# Autodesk Inventor assembly: Cockpit
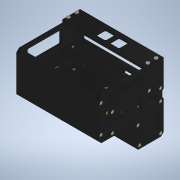
[picture p0: Inventor's stored thumbnail of the model, 180x180]
Saved by Autodesk Inventor 2020 (Build 240168000, 168)
## iProperties
Created: 2022-01-06
Part Number: Cockpit
Document SubType Name: Assembly
Designer: Masato Kubotera
Mass: 580.21 g
Surface Area: 2312.67 cm^2
Volume: 391.499 cm^3
Density: 1.48202 g/cm^3
Author: Masato Kubotera
## Documents named in this file (17)
- C:\Users\MasatoKubotera\Documents\Inventor\OpenPlatform_ver3_0 - prototype\UpperBody\Cockpit\Cockpit.iam
- C:\Users\MasatoKubotera\Documents\Inventor\OpenPlatform_ver3_0 - prototype\ReadyMade\Battery\HP-G830C2800S3.ipt
- C:\Users\MasatoKubotera\Documents\Inventor\OpenPlatform_ver3_0 - prototype\UpperBody\Cockpit\Cockpit_side_frame.ipt
- C:\Users\MasatoKubotera\Documents\Inventor\OpenPlatform_ver3_0 - prototype\UpperBody\Cockpit\Cockpit_battery_back_boor.ipt
- C:\Users\MasatoKubotera\Documents\Inventor\OpenPlatform_ver3_0 - prototype\UpperBody\Cockpit\Cockpit_battery_bottom_frame.ipt
- C:\Users\MasatoKubotera\Documents\Inventor\OpenPlatform_ver3_0 - prototype\UpperBody\Cockpit\Cockpit_battery_front_frame.ipt
- C:\Users\MasatoKubotera\Documents\Inventor\OpenPlatform_ver3_0 - prototype\UpperBody\Cockpit\Cockpit_circuit_board_frame.ipt
- C:\Users\MasatoKubotera\Documents\Inventor\OpenPlatform_ver3_0 - prototype\UpperBody\Cockpit\Cockpit_front_frame.ipt
- C:\Users\MasatoKubotera\Documents\Inventor\OpenPlatform_ver3_0 - prototype\UpperBody\Cockpit\Cockpit_side_frame_MIR.ipt
- C:\Users\MasatoKubotera\Documents\Inventor\OpenPlatform_ver3_0 - prototype\UpperBody\Cockpit\Cockpit_top_frame.ipt
- C:\Users\MasatoKubotera\Documents\Inventor\OpenPlatform_ver3_0 - prototype\UpperBody\Cockpit\Cockpit_carrier_board_frame.ipt
- C:\Users\MasatoKubotera\Documents\Inventor\OpenPlatform_ver3_0 - prototype\UpperBody\Cockpit\Cockpit_back_frame.ipt
- C:\Users\MasatoKubotera\Documents\Inventor\OpenPlatform_ver3_0 - prototype\ReadyMade\InsertNut\UD-43040.ipt
- C:\Users\MasatoKubotera\Documents\Inventor\OpenPlatform_ver3_0 - prototype\ReadyMade\InsertNut\IRU-304SW.ipt
- C:\Users\MasatoKubotera\Documents\Inventor\OpenPlatform_ver3_0 - prototype\ReadyMade\Neodymium_magnet_Phi3_T3.ipt
- C:\Users\MasatoKubotera\Documents\Inventor\OpenPlatform_ver3_0 - prototype\ReadyMade\Screw\M3-8.ipt
- C:\Users\MasatoKubotera\Documents\Inventor\OpenPlatform_ver3_0 - prototype\ReadyMade\Screw\M3-10.ipt
## Components (79 placed, 16 different names)
1. HP-G830C2800S3:1 — メイト:1, メイト:2, メイト:3
2. Cockpit_side_frame:1 — フラッシュ:1, フラッシュ:2, フラッシュ:3, 挿入:1, 挿入:9, 挿入:10, 挿入:33, 挿入:34, 挿入:35, 挿入:49, 挿入:50, 挿入:53, 挿入:54, 挿入:57, 角度:1, 挿入:59, 挿入:61, 挿入:63, 角度:2, 角度:3, 角度:4, 挿入:65, 挿入:66, メイト:3, 挿入:69, 挿入:70, 挿入:73, 挿入:74, 挿入:77, 挿入:79, 挿入:81, 挿入:83, 挿入:85, 挿入:86
3. Cockpit_battery_back_boor:1 — 挿入:27, 挿入:28, 挿入:39, 挿入:40, 挿入:41, 挿入:42, 挿入:43, 挿入:44, 角度:2
4. Cockpit_battery_bottom_frame:1 — 挿入:25, 挿入:26, メイト:1, 角度:4
5. Cockpit_battery_front_frame:1 — 挿入:23, 挿入:24, 角度:3, メイト:2
6. Cockpit_circuit_board_frame:1 — 挿入:3, 挿入:4, 挿入:5, 挿入:6, 挿入:7, 挿入:8, 挿入:17, 挿入:18, 角度:1
7. Cockpit_front_frame:1 — 挿入:13, 挿入:14, 挿入:15, 挿入:16
8. Cockpit_side_frame_MIR:1 — 挿入:2, 挿入:11, 挿入:12, 挿入:36, 挿入:37, 挿入:38, 挿入:51, 挿入:52, 挿入:55, 挿入:56, 挿入:58, 挿入:60, 挿入:62, 挿入:64, 挿入:67, 挿入:68, 挿入:71, 挿入:72, 挿入:75, 挿入:76, 挿入:78, 挿入:80, 挿入:82, 挿入:84, 挿入:87, 挿入:88
9. Cockpit_top_frame:1 — 挿入:45, 挿入:46, 挿入:47, 挿入:48, 挿入:89, 挿入:90, 挿入:91, 挿入:92
10. Cockpit_carrier_board_frame:1 — 挿入:19, 挿入:20, 挿入:22, 挿入:21
11. M3-8:1 — 挿入:69
12. M3-8:2 — 挿入:70
13. M3-8:3 — 挿入:71
14. M3-8:4 — 挿入:72
15. M3-8:5 — 挿入:73
16. M3-8:6 — 挿入:74
17. M3-8:7 — 挿入:75
18. M3-8:8 — 挿入:76
19. M3-8:9 — 挿入:77
20. M3-8:10 — 挿入:78
21. M3-8:11 — 挿入:79
22. M3-8:12 — 挿入:80
23. M3-8:13 — 挿入:81
24. M3-8:14 — 挿入:82
25. M3-8:15 — 挿入:83
26. M3-8:16 — 挿入:84
27. M3-8:17 — 挿入:85
28. M3-8:18 — 挿入:86
29. M3-8:19 — 挿入:87
30. M3-8:20 — 挿入:88
31. M3-10:1 — 挿入:89
32. M3-10:2 — 挿入:90
33. M3-10:3 — 挿入:91
34. M3-10:4 — 挿入:92
35. Cockpit_back_frame:1 — 挿入:29, 挿入:30, 挿入:31, 挿入:32
36. UD-43040:1 — 挿入:1
37. UD-43040:2 — 挿入:2
38. UD-43040:3 — 挿入:3
39. UD-43040:4 — 挿入:4
40. UD-43040:5 — 挿入:5
41. UD-43040:6 — 挿入:6
42. UD-43040:7 — 挿入:7
43. UD-43040:8 — 挿入:8
44. IRU-304SW:1 — 挿入:9, 挿入:45
45. IRU-304SW:2 — 挿入:10, 挿入:46
46. IRU-304SW:3 — 挿入:11, 挿入:47
47. IRU-304SW:4 — 挿入:12, 挿入:48
48. IRU-304SW:5 — 挿入:13, 挿入:49
49. IRU-304SW:6 — 挿入:14, 挿入:50
50. IRU-304SW:7 — 挿入:15, 挿入:51
51. IRU-304SW:8 — 挿入:16, 挿入:52
52. IRU-304SW:9 — 挿入:17, 挿入:57
53. IRU-304SW:10 — 挿入:18, 挿入:58
54. IRU-304SW:11 — 挿入:19, 挿入:53
55. IRU-304SW:12 — 挿入:20, 挿入:54
56. IRU-304SW:13 — 挿入:21, 挿入:55
57. IRU-304SW:14 — 挿入:22, 挿入:56
58. IRU-304SW:15 — 挿入:23, 挿入:59
59. IRU-304SW:16 — 挿入:24, 挿入:60
60. IRU-304SW:17 — 挿入:25, 挿入:61
61. IRU-304SW:18 — 挿入:26, 挿入:62
62. IRU-304SW:19 — 挿入:27, 挿入:63
63. IRU-304SW:20 — 挿入:28, 挿入:64
64. IRU-304SW:21 — 挿入:29, 挿入:65
65. IRU-304SW:22 — 挿入:30, 挿入:66
66. IRU-304SW:23 — 挿入:31, 挿入:67
67. IRU-304SW:24 — 挿入:32, 挿入:68
68. Neodymium_magnet_Phi3_T3:1 — 挿入:33
69. Neodymium_magnet_Phi3_T3:2 — 挿入:34
70. Neodymium_magnet_Phi3_T3:3 — 挿入:35
71. Neodymium_magnet_Phi3_T3:4 — 挿入:36
72. Neodymium_magnet_Phi3_T3:5 — 挿入:37
73. Neodymium_magnet_Phi3_T3:6 — 挿入:38
74. Neodymium_magnet_Phi3_T3:7 — 挿入:39
75. Neodymium_magnet_Phi3_T3:8 — 挿入:40
76. Neodymium_magnet_Phi3_T3:9 — 挿入:41
77. Neodymium_magnet_Phi3_T3:10 — 挿入:42
78. Neodymium_magnet_Phi3_T3:11 — 挿入:43
79. Neodymium_magnet_Phi3_T3:12 — 挿入:44
## Relationships (102: Insert 92, Angle 4, Flush 3, Mate 3)
- フラッシュ:1 [Flush]: Cockpit_side_frame:1
- フラッシュ:2 [Flush] (67.5 mm): Cockpit_side_frame:1
- フラッシュ:3 [Flush]: Cockpit_side_frame:1
- 挿入:1 [Insert]: Cockpit_side_frame:1 ↔ UD-43040:1
- 挿入:2 [Insert]: Cockpit_side_frame_MIR:1 ↔ UD-43040:2
- 挿入:3 [Insert]: Cockpit_circuit_board_frame:1 ↔ UD-43040:3
- 挿入:4 [Insert]: Cockpit_circuit_board_frame:1 ↔ UD-43040:4
- 挿入:5 [Insert]: Cockpit_circuit_board_frame:1 ↔ UD-43040:5
- 挿入:6 [Insert]: Cockpit_circuit_board_frame:1 ↔ UD-43040:6
- 挿入:7 [Insert]: Cockpit_circuit_board_frame:1 ↔ UD-43040:7
- 挿入:8 [Insert]: Cockpit_circuit_board_frame:1 ↔ UD-43040:8
- 挿入:9 [Insert]: Cockpit_side_frame:1 ↔ IRU-304SW:1
- 挿入:10 [Insert]: Cockpit_side_frame:1 ↔ IRU-304SW:2
- 挿入:11 [Insert]: Cockpit_side_frame_MIR:1 ↔ IRU-304SW:3
- 挿入:12 [Insert]: Cockpit_side_frame_MIR:1 ↔ IRU-304SW:4
- 挿入:13 [Insert]: Cockpit_front_frame:1 ↔ IRU-304SW:5
- 挿入:14 [Insert]: Cockpit_front_frame:1 ↔ IRU-304SW:6
- 挿入:15 [Insert]: Cockpit_front_frame:1 ↔ IRU-304SW:7
- 挿入:16 [Insert]: Cockpit_front_frame:1 ↔ IRU-304SW:8
- 挿入:17 [Insert]: Cockpit_circuit_board_frame:1 ↔ IRU-304SW:9
- 挿入:18 [Insert]: Cockpit_circuit_board_frame:1 ↔ IRU-304SW:10
- 挿入:19 [Insert]: Cockpit_carrier_board_frame:1 ↔ IRU-304SW:11
- 挿入:20 [Insert]: Cockpit_carrier_board_frame:1 ↔ IRU-304SW:12
- 挿入:21 [Insert]: Cockpit_carrier_board_frame:1 ↔ IRU-304SW:13
- 挿入:22 [Insert]: Cockpit_carrier_board_frame:1 ↔ IRU-304SW:14
- 挿入:23 [Insert]: Cockpit_battery_front_frame:1 ↔ IRU-304SW:15
- 挿入:24 [Insert]: Cockpit_battery_front_frame:1 ↔ IRU-304SW:16
- 挿入:25 [Insert]: Cockpit_battery_bottom_frame:1 ↔ IRU-304SW:17
- 挿入:26 [Insert]: Cockpit_battery_bottom_frame:1 ↔ IRU-304SW:18
- 挿入:27 [Insert]: Cockpit_battery_back_boor:1 ↔ IRU-304SW:19
- 挿入:28 [Insert]: Cockpit_battery_back_boor:1 ↔ IRU-304SW:20
- 挿入:29 [Insert]: Cockpit_back_frame:1 ↔ IRU-304SW:21
- 挿入:30 [Insert]: Cockpit_back_frame:1 ↔ IRU-304SW:22
- 挿入:31 [Insert]: Cockpit_back_frame:1 ↔ IRU-304SW:23
- 挿入:32 [Insert]: Cockpit_back_frame:1 ↔ IRU-304SW:24
- 挿入:33 [Insert]: Cockpit_side_frame:1 ↔ Neodymium_magnet_Phi3_T3:1
- 挿入:34 [Insert]: Cockpit_side_frame:1 ↔ Neodymium_magnet_Phi3_T3:2
- 挿入:35 [Insert]: Cockpit_side_frame:1 ↔ Neodymium_magnet_Phi3_T3:3
- 挿入:36 [Insert]: Cockpit_side_frame_MIR:1 ↔ Neodymium_magnet_Phi3_T3:4
- 挿入:37 [Insert]: Cockpit_side_frame_MIR:1 ↔ Neodymium_magnet_Phi3_T3:5
- 挿入:38 [Insert]: Cockpit_side_frame_MIR:1 ↔ Neodymium_magnet_Phi3_T3:6
- 挿入:39 [Insert]: Cockpit_battery_back_boor:1 ↔ Neodymium_magnet_Phi3_T3:7
- 挿入:40 [Insert]: Cockpit_battery_back_boor:1 ↔ Neodymium_magnet_Phi3_T3:8
- 挿入:41 [Insert]: Cockpit_battery_back_boor:1 ↔ Neodymium_magnet_Phi3_T3:9
- 挿入:42 [Insert]: Cockpit_battery_back_boor:1 ↔ Neodymium_magnet_Phi3_T3:10
- 挿入:43 [Insert]: Cockpit_battery_back_boor:1 ↔ Neodymium_magnet_Phi3_T3:11
- 挿入:44 [Insert]: Cockpit_battery_back_boor:1 ↔ Neodymium_magnet_Phi3_T3:12
- 挿入:45 [Insert]: Cockpit_top_frame:1 ↔ IRU-304SW:1
- 挿入:46 [Insert]: Cockpit_top_frame:1 ↔ IRU-304SW:2
- 挿入:47 [Insert]: Cockpit_top_frame:1 ↔ IRU-304SW:3
- 挿入:48 [Insert]: Cockpit_top_frame:1 ↔ IRU-304SW:4
- 挿入:49 [Insert]: Cockpit_side_frame:1 ↔ IRU-304SW:5
- 挿入:50 [Insert]: Cockpit_side_frame:1 ↔ IRU-304SW:6
- 挿入:51 [Insert]: Cockpit_side_frame_MIR:1 ↔ IRU-304SW:7
- 挿入:52 [Insert]: Cockpit_side_frame_MIR:1 ↔ IRU-304SW:8
- 挿入:53 [Insert]: Cockpit_side_frame:1 ↔ IRU-304SW:11
- 挿入:54 [Insert]: Cockpit_side_frame:1 ↔ IRU-304SW:12
- 挿入:55 [Insert]: Cockpit_side_frame_MIR:1 ↔ IRU-304SW:13
- 挿入:56 [Insert]: Cockpit_side_frame_MIR:1 ↔ IRU-304SW:14
- 挿入:57 [Insert]: Cockpit_side_frame:1 ↔ IRU-304SW:9
- 挿入:58 [Insert]: Cockpit_side_frame_MIR:1 ↔ IRU-304SW:10
- 角度:1 [Angle] (0 deg): Cockpit_side_frame:1 ↔ Cockpit_circuit_board_frame:1
- 挿入:59 [Insert]: Cockpit_side_frame:1 ↔ IRU-304SW:15
- 挿入:60 [Insert]: Cockpit_side_frame_MIR:1 ↔ IRU-304SW:16
- 挿入:61 [Insert]: Cockpit_side_frame:1 ↔ IRU-304SW:17
- 挿入:62 [Insert]: Cockpit_side_frame_MIR:1 ↔ IRU-304SW:18
- 挿入:63 [Insert]: Cockpit_side_frame:1 ↔ IRU-304SW:19
- 挿入:64 [Insert]: Cockpit_side_frame_MIR:1 ↔ IRU-304SW:20
- 角度:2 [Angle] (0 deg): Cockpit_side_frame:1 ↔ Cockpit_battery_back_boor:1
- 角度:3 [Angle] (0 deg): Cockpit_side_frame:1 ↔ Cockpit_battery_front_frame:1
- 角度:4 [Angle] (0 deg): Cockpit_side_frame:1 ↔ Cockpit_battery_bottom_frame:1
- 挿入:65 [Insert]: Cockpit_side_frame:1 ↔ IRU-304SW:21
- 挿入:66 [Insert]: Cockpit_side_frame:1 ↔ IRU-304SW:22
- 挿入:67 [Insert]: Cockpit_side_frame_MIR:1 ↔ IRU-304SW:23
- 挿入:68 [Insert]: Cockpit_side_frame_MIR:1 ↔ IRU-304SW:24
- メイト:1 [Mate]: HP-G830C2800S3:1 ↔ Cockpit_battery_bottom_frame:1
- メイト:2 [Mate]: HP-G830C2800S3:1 ↔ Cockpit_battery_front_frame:1
- メイト:3 [Mate]: HP-G830C2800S3:1 ↔ Cockpit_side_frame:1
- 挿入:69 [Insert]: Cockpit_side_frame:1 ↔ M3-8:1
- 挿入:70 [Insert]: Cockpit_side_frame:1 ↔ M3-8:2
- 挿入:71 [Insert]: Cockpit_side_frame_MIR:1 ↔ M3-8:3
- 挿入:72 [Insert]: Cockpit_side_frame_MIR:1 ↔ M3-8:4
- 挿入:73 [Insert]: Cockpit_side_frame:1 ↔ M3-8:5
- 挿入:74 [Insert]: Cockpit_side_frame:1 ↔ M3-8:6
- 挿入:75 [Insert]: Cockpit_side_frame_MIR:1 ↔ M3-8:7
- 挿入:76 [Insert]: Cockpit_side_frame_MIR:1 ↔ M3-8:8
- 挿入:77 [Insert]: Cockpit_side_frame:1 ↔ M3-8:9
- 挿入:78 [Insert]: Cockpit_side_frame_MIR:1 ↔ M3-8:10
- 挿入:79 [Insert]: Cockpit_side_frame:1 ↔ M3-8:11
- 挿入:80 [Insert]: Cockpit_side_frame_MIR:1 ↔ M3-8:12
- 挿入:81 [Insert]: Cockpit_side_frame:1 ↔ M3-8:13
- 挿入:82 [Insert]: Cockpit_side_frame_MIR:1 ↔ M3-8:14
- 挿入:83 [Insert]: Cockpit_side_frame:1 ↔ M3-8:15
- 挿入:84 [Insert]: Cockpit_side_frame_MIR:1 ↔ M3-8:16
- 挿入:85 [Insert]: Cockpit_side_frame:1 ↔ M3-8:17
- 挿入:86 [Insert]: Cockpit_side_frame:1 ↔ M3-8:18
- 挿入:87 [Insert]: Cockpit_side_frame_MIR:1 ↔ M3-8:19
- 挿入:88 [Insert]: Cockpit_side_frame_MIR:1 ↔ M3-8:20
- 挿入:89 [Insert]: Cockpit_top_frame:1 ↔ M3-10:1
- 挿入:90 [Insert]: Cockpit_top_frame:1 ↔ M3-10:2
- 挿入:91 [Insert]: Cockpit_top_frame:1 ↔ M3-10:3
- 挿入:92 [Insert]: Cockpit_top_frame:1 ↔ M3-10:4
